# Autodesk Inventor assembly: Linear slides
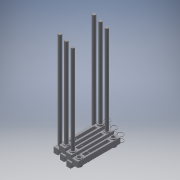
[picture p0: Inventor's stored thumbnail of the model, 180x180]
Saved by Autodesk Inventor 2019 (Build 230136000, 136)
## iProperties
Created: 2019-03-07
Part Number: Linear slides
Document SubType Name: Assembly
Designer: Delta
Author: Delta
## Documents named in this file (4)
- C:\Robotics\2019-20_CAD\Linear Slides\Linear slides.iam
- C:\Robotics\2019-20_CAD\Linear Slides\Block_3-8.ipt
- C:\Robotics\2019-20_CAD\Linear Slides\rod_3-8_12 inch.ipt
- C:\Robotics\COTSParts\Bearings - McMaster\60595K120_FIXED ALIGNMENT  LINEAR BALL BRNG.ipt
## Components (15 placed, 3 different names)
1. Block_3-8:1 — Mate:3, Mate:4, Mate:9, Mate:11, Mate:13, Mate:14, Mate:19, Mate:20
2. Block_3-8:2 — Mate:5, Mate:6, Mate:10, Mate:12, Mate:17, Mate:18, Mate:23, Mate:24
3. Block_3-8:3 — Mate:1, Mate:2, Mate:7, Mate:8, Mate:15, Mate:16, Mate:21, Mate:22
4. rod_3-8_12 inch:1 — Mate:4, Mate:11, Mate:27
5. rod_3-8_12 inch:2 — Mate:5, Mate:10
6. rod_3-8_12 inch:3 — Mate:3, Mate:9, Mate:28
7. rod_3-8_12 inch:4 — Mate:6, Mate:12
8. rod_3-8_12 inch:5 — Mate:1, Mate:8, Mate:25
9. rod_3-8_12 inch:6 — Mate:2, Mate:7, Mate:26
10. 60595K120_FIXED ALIGNMENT  LINEAR BALL BRNG:1 — Mate:16, Mate:22
11. 60595K120_FIXED ALIGNMENT  LINEAR BALL BRNG:2 — Mate:13, Mate:19, Mate:26
12. 60595K120_FIXED ALIGNMENT  LINEAR BALL BRNG:3 — Mate:15, Mate:21
13. 60595K120_FIXED ALIGNMENT  LINEAR BALL BRNG:4 — Mate:14, Mate:20, Mate:25
14. 60595K120_FIXED ALIGNMENT  LINEAR BALL BRNG:5 — Mate:17, Mate:23, Mate:28
15. 60595K120_FIXED ALIGNMENT  LINEAR BALL BRNG:6 — Mate:18, Mate:24, Mate:27
## Relationships (28: Mate 28)
- Mate:1: Block_3-8:3 ↔ rod_3-8_12 inch:5
- Mate:2: Block_3-8:3 ↔ rod_3-8_12 inch:6
- Mate:3: Block_3-8:1 ↔ rod_3-8_12 inch:3
- Mate:4: Block_3-8:1 ↔ rod_3-8_12 inch:1
- Mate:5: Block_3-8:2 ↔ rod_3-8_12 inch:2
- Mate:6: Block_3-8:2 ↔ rod_3-8_12 inch:4
- Mate:7: Block_3-8:3 ↔ rod_3-8_12 inch:6
- Mate:8: Block_3-8:3 ↔ rod_3-8_12 inch:5
- Mate:9: Block_3-8:1 ↔ rod_3-8_12 inch:3
- Mate:10: Block_3-8:2 ↔ rod_3-8_12 inch:2
- Mate:11: Block_3-8:1 ↔ rod_3-8_12 inch:1
- Mate:12: Block_3-8:2 ↔ rod_3-8_12 inch:4
- Mate:13: Block_3-8:1 ↔ 60595K120_FIXED ALIGNMENT  LINEAR BALL BRNG:2
- Mate:14: Block_3-8:1 ↔ 60595K120_FIXED ALIGNMENT  LINEAR BALL BRNG:4
- Mate:15: Block_3-8:3 ↔ 60595K120_FIXED ALIGNMENT  LINEAR BALL BRNG:3
- Mate:16: Block_3-8:3 ↔ 60595K120_FIXED ALIGNMENT  LINEAR BALL BRNG:1
- Mate:17: Block_3-8:2 ↔ 60595K120_FIXED ALIGNMENT  LINEAR BALL BRNG:5
- Mate:18: Block_3-8:2 ↔ 60595K120_FIXED ALIGNMENT  LINEAR BALL BRNG:6
- Mate:19: Block_3-8:1 ↔ 60595K120_FIXED ALIGNMENT  LINEAR BALL BRNG:2
- Mate:20: Block_3-8:1 ↔ 60595K120_FIXED ALIGNMENT  LINEAR BALL BRNG:4
- Mate:21: Block_3-8:3 ↔ 60595K120_FIXED ALIGNMENT  LINEAR BALL BRNG:3
- Mate:22: Block_3-8:3 ↔ 60595K120_FIXED ALIGNMENT  LINEAR BALL BRNG:1
- Mate:23: Block_3-8:2 ↔ 60595K120_FIXED ALIGNMENT  LINEAR BALL BRNG:5
- Mate:24: Block_3-8:2 ↔ 60595K120_FIXED ALIGNMENT  LINEAR BALL BRNG:6
- Mate:25: rod_3-8_12 inch:5 ↔ 60595K120_FIXED ALIGNMENT  LINEAR BALL BRNG:4
- Mate:26: rod_3-8_12 inch:6 ↔ 60595K120_FIXED ALIGNMENT  LINEAR BALL BRNG:2
- Mate:27: rod_3-8_12 inch:1 ↔ 60595K120_FIXED ALIGNMENT  LINEAR BALL BRNG:6
- Mate:28: rod_3-8_12 inch:3 ↔ 60595K120_FIXED ALIGNMENT  LINEAR BALL BRNG:5
